# Autodesk Inventor assembly: Drivetrain Side
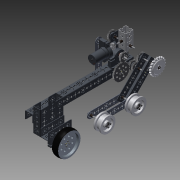
[picture p0: Inventor's stored thumbnail of the model, 180x180]
Saved by Autodesk Inventor 2015 (Build 190159000, 159)
## iProperties
Created: 2015-09-28
Part Number: Drivetrain Side
Document SubType Name: Assembly
Designer: Jing-Chen
Author: Jing-Chen
## Documents named in this file (22)
- C:\Users\Jing-Chen\Desktop\Bionic Hybrids 2016\Bionic-Hybrids\CAD\Drivetrain\Sub-Assemblies\Drivetrain Side.iam
- C:\Users\Jing-Chen\Desktop\Bionic Hybrids 2016\Bionic-Hybrids\Stock\Bracket-U25 - 739069.ipt
- C:\Users\Jing-Chen\Desktop\Bionic Hybrids 2016\Bionic-Hybrids\CAD\Drivetrain\Sub-Assemblies\Wheel Assembly.iam
- C:\Users\Jing-Chen\Desktop\Bionic Hybrids 2016\Bionic-Hybrids\CAD\Drivetrain\Sub-Assemblies\Track Frame Assembly.iam
- C:\Users\Jing-Chen\Desktop\Bionic Hybrids 2016\Bionic-Hybrids\Stock\Bearing-Thrust - 739091.ipt
- C:\Users\Jing-Chen\Desktop\Bionic Hybrids 2016\Bionic-Hybrids\Stock\Motor Mount - 739089.ipt
- C:\Users\Jing-Chen\Desktop\Bionic Hybrids 2016\Bionic-Hybrids\Stock\Bracket-U5 - 739066.ipt
- C:\Users\Jing-Chen\Desktop\Bionic Hybrids 2016\Bionic-Hybrids\CAD\General\Modified Parts\Movable Motor.iam
- C:\Users\Jing-Chen\Desktop\Bionic Hybrids 2016\Bionic-Hybrids\Stock\Gear-80 tooth - 731901.ipt
- C:\Users\Jing-Chen\Desktop\Bionic Hybrids 2016\Bionic-Hybrids\Stock\Plate-2x1 Long - 739061.ipt
- C:\Users\Jing-Chen\Desktop\Bionic Hybrids 2016\Bionic-Hybrids\Stock\Shaft Collar-Setscrew, Axle, Mountable - 739079.iam
- C:\Users\Jing-Chen\Desktop\Bionic Hybrids 2016\Bionic-Hybrids\Stock\Screw 0.5in - 739097.ipt
- C:\Users\Jing-Chen\Desktop\Bionic Hybrids 2016\Bionic-Hybrids\Stock\Shaft Collar-Setscrew, Axle, Mountable - 739172.iam
- C:\Users\Jing-Chen\Desktop\Bionic Hybrids 2016\Bionic-Hybrids\Stock\Gear-40 tooth - 731901.ipt
- C:\Users\Jing-Chen\Desktop\Bionic Hybrids 2016\Bionic-Hybrids\Stock\Nut-Locking - 739094.ipt
- C:\Users\Jing-Chen\Desktop\Bionic Hybrids 2016\Bionic-Hybrids\CAD\General\40-tooth Gear Assembly.iam
- C:\Users\Jing-Chen\Desktop\Bionic Hybrids 2016\Bionic-Hybrids\Stock\Plate-9x1 - 739272.ipt
- C:\Users\Jing-Chen\Desktop\Bionic Hybrids 2016\Bionic-Hybrids\New Stock\Worm Gear Abstract.iam
- C:\Users\Jing-Chen\Desktop\Bionic Hybrids 2016\Bionic-Hybrids\Stock\Shaft Collar-Setscrew, Axle - 739092.iam
- C:\Users\Jing-Chen\Desktop\Bionic Hybrids 2016\Bionic-Hybrids\CAD\General\Modified Parts\55mm axle.ipt
- C:\Users\Jing-Chen\Desktop\Bionic Hybrids 2016\Bionic-Hybrids\Stock\Axle-100mm - 739088.ipt
- C:\Users\Jing-Chen\Desktop\Bionic Hybrids 2016\Bionic-Hybrids\CAD\General\Modified Parts\Cut 100mm axle.ipt
## Components (54 placed, 21 different names)
1. Track Frame Assembly:1 [sub-assembly] — Mate:33, Mate:36, Rotation:2, Mate:157, Mate:160, Angle:11
2. Bearing-Thrust - 739091:1 — Mate:33, Mate:36, Mate:60, Mate:61
3. Motor Mount - 739089:1 — Mate:40, Flush:1, Mate:51, Mate:52, Mate:53
4. Wheel Assembly:1 [sub-assembly] — Angle:2, Mate:41, Flush:2
5. Movable Motor:1 [sub-assembly] — Mate:40, Flush:1, Angle:1, Angle:2, Mate:41, Flush:2
6. Bracket-U5 - 739066:1 — Mate:44, Mate:46, Mate:47, Mate:51, Mate:52, Mate:53
7. Bracket-U5 - 739066:2 — Mate:44, Mate:46, Mate:47, Mate:54, Mate:55, Mate:56
8. Bracket-U5 - 739066:3 — Mate:57, Mate:58, Mate:59
9. Bracket-U25 - 739069:1 — Mate:54, Mate:55, Mate:56, Mate:57, Mate:58, Mate:59, Mate:60, Mate:61, Mate:62, Angle:3, Mate:81, Mate:96, Mate:97, Mate:126, Mate:128, Mate:129, Mate:130, Mate:131, Mate:132, Mate:133, Mate:135, Mate:137, Mate:140, Mate:141, Mate:165, Mate:170, Mate:173
10. Movable Motor:2 [sub-assembly] — Mate:64, Flush:3, Angle:4, Angle:5, Mate:108
11. Motor Mount - 739089:2 — Mate:62, Angle:3, Mate:64, Flush:3, Mate:82, Mate:83, Mate:116
12. Plate-2x1 Long - 739061:2 — Mate:81, Mate:82, Mate:83, Mate:116
13. Shaft Collar-Setscrew, Axle, Mountable - 739079:1 [sub-assembly] — Angle:5, Mate:104, Mate:105, Mate:106, Mate:107, Mate:108, Mate:109, Mate:111
14. Screw 0.5in - 739097:1 — Mate:105, Mate:110, Mate:113
15. Screw 0.5in - 739097:2 — Mate:107, Mate:112
16. Screw 0.5in - 739097:3 — Mate:104, Mate:114
17. Screw 0.5in - 739097:4 — Mate:106, Mate:115
18. Bearing-Thrust - 739091:2 — Mate:96, Mate:97, Mate:100
19. Shaft Collar-Setscrew, Axle, Mountable - 739172:1 [sub-assembly] — Mate:100, Mate:102, Mate:103, Mate:121, Mate:122, Mate:123, Mate:124, Mate:179
20. Gear-80 tooth - 731901:2 — Mate:102, Mate:103, Flush:4, Rotation:1, Rotation:2, Mate:117, Mate:118, Mate:119, Mate:120, Mate:178, Flush:7
21. Gear-40 tooth - 731901:1 — Mate:109, Mate:110, Mate:111, Mate:112, Mate:113, Mate:114, Mate:115, Flush:4, Rotation:1
22. Screw 0.5in - 739097:5 — Mate:118, Mate:122
23. Screw 0.5in - 739097:6 — Mate:117, Mate:121
24. Screw 0.5in - 739097:7 — Mate:119, Mate:123
25. Screw 0.5in - 739097:8 — Mate:120, Mate:124, Mate:178
26. Bearing-Thrust - 739091:3 — Mate:126, Mate:128, Mate:177, Mate:181
27. Bracket-U5 - 739066:4 — Mate:129, Mate:142, Mate:143, Mate:144, Mate:145, Mate:146, Mate:148, Mate:147, Mate:149, Mate:150, Mate:151, Mate:152, Mate:153, Mate:154, Mate:174, Mate:175, Mate:176
28. Screw 0.5in - 739097:9 — Mate:133, Mate:134, Mate:144
29. Screw 0.5in - 739097:10 — Mate:131, Mate:136, Mate:143
30. Screw 0.5in - 739097:11 — Mate:130, Mate:139, Mate:142, Mate:146
31. Screw 0.5in - 739097:12 — Mate:132, Mate:138, Mate:145
32. Nut-Locking - 739094:1 — Mate:136, Mate:137
33. Nut-Locking - 739094:2 — Mate:134, Mate:135
34. Nut-Locking - 739094:3 — Mate:139, Mate:140
35. Nut-Locking - 739094:4 — Mate:138, Mate:141
36. Bearing-Thrust - 739091:4 — Mate:147, Mate:148, Mate:158, Mate:160
37. Bearing-Thrust - 739091:5 — Mate:149, Mate:150, Mate:182, Mate:184
38. Bearing-Thrust - 739091:6 — Mate:151, Mate:152, Mate:187, Mate:189
39. Bearing-Thrust - 739091:7 — Mate:153, Mate:154, Mate:186
40. 40-tooth Gear Assembly:1 [sub-assembly] — Mate:157, Mate:158, Angle:11, Rotation:4
41. 40-tooth Gear Assembly:2 [sub-assembly] — Mate:183, Mate:184, Flush:8, Rotation:3, Rotation:4
42. 40-tooth Gear Assembly:3 [sub-assembly] — Mate:188, Mate:189, Flush:9, Rotation:3, Angle:14
43. Movable Motor:3 [sub-assembly] — Mate:169, Flush:6, Angle:7, Angle:12, Mate:191, Flush:10, Mate:192
44. Motor Mount - 739089:3 — Mate:169, Flush:6, Mate:171, Angle:10, Mate:172
45. Plate-9x1 - 739272:1 — Mate:165, Mate:170, Mate:171, Angle:10, Mate:172, Mate:173
46. Worm Gearbox, Ratio 20:1 [sub-assembly] — Mate:174, Mate:175, Mate:176, Mate:190
47. 55mm axle:1 — Mate:177, Mate:179, Flush:7, Mate:180
48. Shaft Collar-Setscrew, Axle - 739092:1 [sub-assembly] — Mate:180, Mate:181
49. Shaft Collar-Setscrew, Axle - 739092:2 [sub-assembly] — Mate:185, Mate:186
50. 55mm axle:2 — Mate:182, Mate:183, Flush:8, Mate:185
51. Axle-100mm - 739088:1 — Mate:187, Mate:188, Flush:9, Rotation:5, Angle:14
52. Shaft Collar-Setscrew, Axle, Mountable - 739079:2 [sub-assembly] — Angle:12, Mate:191, Flush:10, Mate:194, Mate:195
53. Shaft Collar-Setscrew, Axle, Mountable - 739172:2 [sub-assembly] — Angle:13, Mate:193, Mate:194, Mate:195
54. Cut 100mm axle:1 — Mate:190, Mate:192, Angle:13, Mate:193, Rotation:5
## Relationships (133: Mate 108, Angle 11, Flush 9, RelateRotation 5)
- Mate:33: Track Frame Assembly:1 ↔ Bearing-Thrust - 739091:1
- Mate:36: Track Frame Assembly:1 ↔ Bearing-Thrust - 739091:1
- Mate:40: Motor Mount - 739089:1 ↔ Movable Motor:1
- Flush:1: Motor Mount - 739089:1 ↔ Movable Motor:1
- Angle:1 (180 deg): Movable Motor:1
- Angle:2 (180 deg): Wheel Assembly:1 ↔ Movable Motor:1
- Mate:41: Wheel Assembly:1 ↔ Movable Motor:1
- Flush:2: Wheel Assembly:1 ↔ Movable Motor:1
- Mate:44: Bracket-U5 - 739066:1 ↔ Bracket-U5 - 739066:2
- Mate:46: Bracket-U5 - 739066:1 ↔ Bracket-U5 - 739066:2
- Mate:47: Bracket-U5 - 739066:1 ↔ Bracket-U5 - 739066:2
- Mate:51: Motor Mount - 739089:1 ↔ Bracket-U5 - 739066:1
- Mate:52: Motor Mount - 739089:1 ↔ Bracket-U5 - 739066:1
- Mate:53: Motor Mount - 739089:1 ↔ Bracket-U5 - 739066:1
- Mate:54: Bracket-U5 - 739066:2 ↔ Bracket-U25 - 739069:1
- Mate:55: Bracket-U5 - 739066:2 ↔ Bracket-U25 - 739069:1
- Mate:56: Bracket-U5 - 739066:2 ↔ Bracket-U25 - 739069:1
- Mate:57: Bracket-U5 - 739066:3 ↔ Bracket-U25 - 739069:1
- Mate:58: Bracket-U5 - 739066:3 ↔ Bracket-U25 - 739069:1
- Mate:59: Bracket-U5 - 739066:3 ↔ Bracket-U25 - 739069:1
- Mate:60: Bearing-Thrust - 739091:1 ↔ Bracket-U25 - 739069:1
- Mate:61: Bearing-Thrust - 739091:1 ↔ Bracket-U25 - 739069:1
- Mate:62: Bracket-U25 - 739069:1 ↔ Motor Mount - 739089:2
- Angle:3 (0 deg): Bracket-U25 - 739069:1 ↔ Motor Mount - 739089:2
- Mate:64: Movable Motor:2 ↔ Motor Mount - 739089:2
- Flush:3: Movable Motor:2 ↔ Motor Mount - 739089:2
- Angle:4 (190 deg): Movable Motor:2
- Mate:81: Bracket-U25 - 739069:1 ↔ Plate-2x1 Long - 739061:2
- Mate:82: Motor Mount - 739089:2 ↔ Plate-2x1 Long - 739061:2
- Mate:83: Motor Mount - 739089:2 ↔ Plate-2x1 Long - 739061:2
- Angle:5 (180 deg): Movable Motor:2 ↔ Shaft Collar-Setscrew, Axle, Mountable - 739079:1
- Mate:96: Bracket-U25 - 739069:1 ↔ Bearing-Thrust - 739091:2
- Mate:97: Bracket-U25 - 739069:1 ↔ Bearing-Thrust - 739091:2
- Mate:100: Bearing-Thrust - 739091:2 ↔ Shaft Collar-Setscrew, Axle, Mountable - 739172:1
- Mate:102: Shaft Collar-Setscrew, Axle, Mountable - 739172:1 ↔ Gear-80 tooth - 731901:2
- Mate:103: Shaft Collar-Setscrew, Axle, Mountable - 739172:1 ↔ Gear-80 tooth - 731901:2
- Mate:104: Shaft Collar-Setscrew, Axle, Mountable - 739079:1 ↔ Screw 0.5in - 739097:3
- Mate:105: Shaft Collar-Setscrew, Axle, Mountable - 739079:1 ↔ Screw 0.5in - 739097:1
- Mate:106: Shaft Collar-Setscrew, Axle, Mountable - 739079:1 ↔ Screw 0.5in - 739097:4
- Mate:107: Shaft Collar-Setscrew, Axle, Mountable - 739079:1 ↔ Screw 0.5in - 739097:2
- Mate:108: Movable Motor:2 ↔ Shaft Collar-Setscrew, Axle, Mountable - 739079:1
- Mate:109: Shaft Collar-Setscrew, Axle, Mountable - 739079:1 ↔ Gear-40 tooth - 731901:1
- Mate:110: Screw 0.5in - 739097:1 ↔ Gear-40 tooth - 731901:1
- Mate:111: Shaft Collar-Setscrew, Axle, Mountable - 739079:1 ↔ Gear-40 tooth - 731901:1
- Mate:112: Screw 0.5in - 739097:2 ↔ Gear-40 tooth - 731901:1
- Mate:113: Screw 0.5in - 739097:1 ↔ Gear-40 tooth - 731901:1
- Mate:114: Screw 0.5in - 739097:3 ↔ Gear-40 tooth - 731901:1
- Mate:115: Screw 0.5in - 739097:4 ↔ Gear-40 tooth - 731901:1
- Mate:116: Motor Mount - 739089:2 ↔ Plate-2x1 Long - 739061:2
- Flush:4: Gear-80 tooth - 731901:2 ↔ Gear-40 tooth - 731901:1
- Rotation:1 [RelateRotation] (0.5 ul): Gear-80 tooth - 731901:2 ↔ Gear-40 tooth - 731901:1
- Rotation:2 [RelateRotation] (2 ul): Track Frame Assembly:1 ↔ Gear-80 tooth - 731901:2
- Mate:117: Gear-80 tooth - 731901:2 ↔ Screw 0.5in - 739097:6
- Mate:118: Gear-80 tooth - 731901:2 ↔ Screw 0.5in - 739097:5
- Mate:119: Gear-80 tooth - 731901:2 ↔ Screw 0.5in - 739097:7
- Mate:120: Gear-80 tooth - 731901:2 ↔ Screw 0.5in - 739097:8
- Mate:121: Shaft Collar-Setscrew, Axle, Mountable - 739172:1 ↔ Screw 0.5in - 739097:6
- Mate:122: Shaft Collar-Setscrew, Axle, Mountable - 739172:1 ↔ Screw 0.5in - 739097:5
- Mate:123: Shaft Collar-Setscrew, Axle, Mountable - 739172:1 ↔ Screw 0.5in - 739097:7
- Mate:124: Shaft Collar-Setscrew, Axle, Mountable - 739172:1 ↔ Screw 0.5in - 739097:8
- Mate:126: Bracket-U25 - 739069:1 ↔ Bearing-Thrust - 739091:3
- Mate:128: Bracket-U25 - 739069:1 ↔ Bearing-Thrust - 739091:3
- Mate:129: Bracket-U25 - 739069:1 ↔ Bracket-U5 - 739066:4
- Mate:130: Bracket-U25 - 739069:1 ↔ Screw 0.5in - 739097:11
- Mate:131: Bracket-U25 - 739069:1 ↔ Screw 0.5in - 739097:10
- Mate:132: Bracket-U25 - 739069:1 ↔ Screw 0.5in - 739097:12
- Mate:133: Bracket-U25 - 739069:1 ↔ Screw 0.5in - 739097:9
- Mate:134: Screw 0.5in - 739097:9 ↔ Nut-Locking - 739094:2
- Mate:135: Bracket-U25 - 739069:1 ↔ Nut-Locking - 739094:2
- Mate:136: Screw 0.5in - 739097:10 ↔ Nut-Locking - 739094:1
- Mate:137: Bracket-U25 - 739069:1 ↔ Nut-Locking - 739094:1
- Mate:138: Screw 0.5in - 739097:12 ↔ Nut-Locking - 739094:4
- Mate:139: Screw 0.5in - 739097:11 ↔ Nut-Locking - 739094:3
- Mate:140: Bracket-U25 - 739069:1 ↔ Nut-Locking - 739094:3
- Mate:141: Bracket-U25 - 739069:1 ↔ Nut-Locking - 739094:4
- Mate:142: Bracket-U5 - 739066:4 ↔ Screw 0.5in - 739097:11
- Mate:143: Bracket-U5 - 739066:4 ↔ Screw 0.5in - 739097:10
- Mate:144: Bracket-U5 - 739066:4 ↔ Screw 0.5in - 739097:9
- Mate:145: Bracket-U5 - 739066:4 ↔ Screw 0.5in - 739097:12
- Mate:146: Bracket-U5 - 739066:4 ↔ Screw 0.5in - 739097:11
- Mate:147: Bracket-U5 - 739066:4 ↔ Bearing-Thrust - 739091:4
- Mate:148: Bracket-U5 - 739066:4 ↔ Bearing-Thrust - 739091:4
- Mate:149: Bracket-U5 - 739066:4 ↔ Bearing-Thrust - 739091:5
- Mate:150: Bracket-U5 - 739066:4 ↔ Bearing-Thrust - 739091:5
- Mate:151: Bracket-U5 - 739066:4 ↔ Bearing-Thrust - 739091:6
- Mate:152: Bracket-U5 - 739066:4 ↔ Bearing-Thrust - 739091:6
- Mate:153: Bracket-U5 - 739066:4 ↔ Bearing-Thrust - 739091:7
- Mate:154: Bracket-U5 - 739066:4 ↔ Bearing-Thrust - 739091:7
- Mate:157: Track Frame Assembly:1 ↔ 40-tooth Gear Assembly:1
- Mate:158: Bearing-Thrust - 739091:4 ↔ 40-tooth Gear Assembly:1
- Mate:160: Track Frame Assembly:1 ↔ Bearing-Thrust - 739091:4
- Mate:165: Bracket-U25 - 739069:1 ↔ Plate-9x1 - 739272:1
- Mate:169: Movable Motor:3 ↔ Motor Mount - 739089:3
- Flush:6: Movable Motor:3 ↔ Motor Mount - 739089:3
- Angle:7 (180 deg): Movable Motor:3
- Mate:170: Bracket-U25 - 739069:1 ↔ Plate-9x1 - 739272:1
- Mate:171: Motor Mount - 739089:3 ↔ Plate-9x1 - 739272:1
- Angle:10 (180 deg): Motor Mount - 739089:3 ↔ Plate-9x1 - 739272:1
- Mate:172: Motor Mount - 739089:3 ↔ Plate-9x1 - 739272:1
- Mate:173: Bracket-U25 - 739069:1 ↔ Plate-9x1 - 739272:1
- Mate:174: Bracket-U5 - 739066:4 ↔ Worm Gearbox, Ratio 20:1
- Mate:175: Bracket-U5 - 739066:4 ↔ Worm Gearbox, Ratio 20:1
- Mate:176: Bracket-U5 - 739066:4 ↔ Worm Gearbox, Ratio 20:1
- Mate:177: Bearing-Thrust - 739091:3 ↔ 55mm axle:1
- Mate:178: Gear-80 tooth - 731901:2 ↔ Screw 0.5in - 739097:8
- Mate:179: Shaft Collar-Setscrew, Axle, Mountable - 739172:1 ↔ 55mm axle:1
- Flush:7: Gear-80 tooth - 731901:2 ↔ 55mm axle:1
- Mate:180: 55mm axle:1 ↔ Shaft Collar-Setscrew, Axle - 739092:1
- Mate:181: Bearing-Thrust - 739091:3 ↔ Shaft Collar-Setscrew, Axle - 739092:1
- Mate:182: Bearing-Thrust - 739091:5 ↔ 55mm axle:2
- Mate:183: 40-tooth Gear Assembly:2 ↔ 55mm axle:2
- Mate:184: Bearing-Thrust - 739091:5 ↔ 40-tooth Gear Assembly:2
- Flush:8: 40-tooth Gear Assembly:2 ↔ 55mm axle:2
- Angle:11 (180 deg): Track Frame Assembly:1 ↔ 40-tooth Gear Assembly:1
- Mate:185: Shaft Collar-Setscrew, Axle - 739092:2 ↔ 55mm axle:2
- Mate:186: Bearing-Thrust - 739091:7 ↔ Shaft Collar-Setscrew, Axle - 739092:2
- Mate:187: Bearing-Thrust - 739091:6 ↔ Axle-100mm - 739088:1
- Mate:188: 40-tooth Gear Assembly:3 ↔ Axle-100mm - 739088:1
- Mate:189: Bearing-Thrust - 739091:6 ↔ 40-tooth Gear Assembly:3
- Flush:9: 40-tooth Gear Assembly:3 ↔ Axle-100mm - 739088:1
- Rotation:3 [RelateRotation] (1 ul): 40-tooth Gear Assembly:2 ↔ 40-tooth Gear Assembly:3
- Rotation:4 [RelateRotation] (1 ul): 40-tooth Gear Assembly:1 ↔ 40-tooth Gear Assembly:2
- Mate:190: Worm Gearbox, Ratio 20:1 ↔ Cut 100mm axle:1
- Angle:12 (180 deg): Movable Motor:3 ↔ Shaft Collar-Setscrew, Axle, Mountable - 739079:2
- Mate:191: Movable Motor:3 ↔ Shaft Collar-Setscrew, Axle, Mountable - 739079:2
- Flush:10: Movable Motor:3 ↔ Shaft Collar-Setscrew, Axle, Mountable - 739079:2
- Mate:192: Movable Motor:3 ↔ Cut 100mm axle:1
- Angle:13 (180 deg): Shaft Collar-Setscrew, Axle, Mountable - 739172:2 ↔ Cut 100mm axle:1
- Mate:193: Shaft Collar-Setscrew, Axle, Mountable - 739172:2 ↔ Cut 100mm axle:1
- Mate:194: Shaft Collar-Setscrew, Axle, Mountable - 739079:2 ↔ Shaft Collar-Setscrew, Axle, Mountable - 739172:2
- Mate:195: Shaft Collar-Setscrew, Axle, Mountable - 739079:2 ↔ Shaft Collar-Setscrew, Axle, Mountable - 739172:2
- Rotation:5 [RelateRotation] (0.05 ul): Axle-100mm - 739088:1 ↔ Cut 100mm axle:1
- Angle:14 (180 deg): 40-tooth Gear Assembly:3 ↔ Axle-100mm - 739088:1
